# Autodesk Inventor assembly: 28BYJ-48 stepper motor
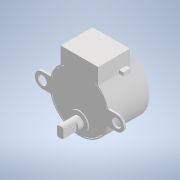
[picture p0: Inventor's stored thumbnail of the model, 180x180]
Saved by Autodesk Inventor 2020.2 (Build 242310000, 310)
## iProperties
Created: 2020-02-18
Part Number: 28BYJ-48 stepper motor
Description: STEP AP203
Document SubType Name: Assembly
Designer: Amaan Khalid
Title: 5V Stepper Motor.stp
Revision Number: NONE
Preprocessor: Spatial InterOp 3D
## Documents named in this file (6)
- C:\Users\Amaan Khalid\Desktop\Robotic Arm project\My parts\Components Cads\28BYJ-48 stepper motor.iam
- C:\Users\Amaan Khalid\Desktop\Część1.ipt
- C:\Users\Amaan Khalid\Desktop\Część2.ipt
- C:\Users\Amaan Khalid\Desktop\Część3.ipt
- C:\Users\Amaan Khalid\Desktop\Część4.ipt
- C:\Users\Amaan Khalid\Desktop\Część11.ipt
## Components (5 placed, 5 different names)
1. Cz___1 — Mate:1, Mate:3
2. Cz___2 — Rotational:1, Mate:1, Mate:2
3. Cz___3 — Mate:2, Mate:3
4. Cz___4 — Rotational:1
5. Cz___11
## Relationships (4: Mate 3, RevoluteJoint 1)
- Rotational:1 [RevoluteJoint]: Cz___2 ↔ Cz___4
- Mate:1: Cz___1 ↔ Cz___2
- Mate:2: Cz___2 ↔ Cz___3
- Mate:3: Cz___1 ↔ Cz___3
